# Autodesk Inventor assembly: Shoulder_support_assembly_without_mount
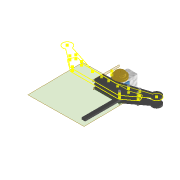
[picture p0: Inventor's stored thumbnail of the model, 180x180]
Saved by Autodesk Inventor 2022 (Build 260153000, 153)
## iProperties
Created: 2022-08-23
Part Number: Shoulder_support_assembly_without_mount
Document SubType Name: Assembly
Designer: dell
Mass: 215.1 g
Surface Area: 1120.32 cm^2
Volume: 215.1 cm^3
Author: dell
## Documents named in this file (11)
- D:\xxxx\Uni\Part IV\MECHENG_700\Part_IV_project_CAD\Bird_skeleton_prototypes\Wing_drone_V1\Bird_wing_V2\Wing_shoulder\Shoulder_support_assembly_without_mount.iam
- D:\xxxx\Uni\Part IV\MECHENG_700\Part_IV_project_CAD\Bird_skeleton_prototypes\Wing_drone_V1\Bird_wing_V2\Wing_shoulder\Vertical_bar.ipt
- D:\xxxx\Uni\Part IV\MECHENG_700\Part_IV_project_CAD\Bird_skeleton_prototypes\Wing_drone_V1\Bird_wing_V2\Wing_shoulder\Horizontal_bar_V2.ipt
- D:\xxxx\Uni\Part IV\MECHENG_700\Part_IV_project_CAD\Bird_skeleton_prototypes\Wing_drone_V1\Bird_wing_V2\Motor_pulley_assembly.iam
- D:\xxxx\Uni\Part IV\MECHENG_700\Part_IV_project_CAD\Bird_skeleton_prototypes\Wing_drone_V1\Bird_wing_V2\Wing_shoulder\Horizontal_bar_support_V2.ipt
- D:\xxxx\Uni\Part IV\MECHENG_700\Part_IV_project_CAD\Bird_skeleton_prototypes\Wing_drone_V1\Bird_wing_V2\Wing_shoulder\Horizontal_bar_spacer.ipt
- D:\xxxx\Uni\Part IV\MECHENG_700\Part_IV_project_CAD\Bird_skeleton_prototypes\Wing_drone_V1\Bird_wing_V2\Wing_shoulder\Horizontal_bar_p2_V2.ipt
- D:\xxxx\Uni\Part IV\MECHENG_700\Part_IV_project_CAD\Bird_skeleton_prototypes\Wing_drone_V1\Bird_wing_V2\Wing_shoulder\Horizontal_bar_spacer_small.ipt
- D:\xxxx\Uni\Part IV\MECHENG_700\Part_IV_project_CAD\Bird_skeleton_prototypes\Wing_drone_V1\Bird_wing_V2\M3_shoulder_bolt.ipt
- D:\xxxx\Uni\Part IV\MECHENG_700\Part_IV_project_CAD\Bird_skeleton_prototypes\Wing_drone_V1\Bird_wing_V2\M3_nut.ipt
- D:\xxxx\Uni\Part IV\MECHENG_700\Part_IV_project_CAD\Bird_skeleton_prototypes\Wing_drone_V1\Bird_wing_V2\M2.5_bolt.ipt
## Components (33 placed, 10 different names)
1. Vertical_bar:1 — Mate:5
2. Vertical_bar:4 — Mate:5, Mate:16, Mate:26, Mate:27
3. Horizontal_bar_V2:1 — Mate:16, Mate:19, Mate:20, Mate:21, Mate:23, Mate:24, Mate:25, Mate:28, Mate:30, Mate:52, Mate:53, Mate:54, Mate:55, Mate:80, Mate:81, Mate:82, Mate:83
4. Motor_pulley_assembly:3 [sub-assembly] — Mate:19, Mate:20, Mate:21, Mate:22, Mate:88, Mate:89, Mate:90, Mate:91, Mate:92, Mate:93, Mate:94, Mate:95
5. Motor_pulley_assembly:4 [sub-assembly] — Mate:23, Mate:24, Mate:25
6. Horizontal_bar_support_V2:2 — Mate:26, Mate:27, Mate:29, Mate:31, Mate:41, Mate:42, Mate:43, Mate:56, Mate:57, Mate:58, Mate:59, Mate:60, Mate:61, Mate:62, Mate:63, Mate:64, Mate:65, Mate:66, Mate:67, Mate:84, Mate:85, Mate:86, Mate:87
7. Horizontal_bar_spacer:4 — Mate:30, Mate:31
8. Horizontal_bar_spacer:5 — Mate:28, Mate:29
9. Horizontal_bar_p2_V2:1 — Mate:41, Mate:42, Mate:43, Mate:44, Mate:45, Mate:46, Mate:47, Mate:68, Mate:69, Mate:70, Mate:71, Mate:72, Mate:73, Mate:74, Mate:75
10. Horizontal_bar_spacer_small:1 — Mate:44, Mate:45
11. Horizontal_bar_spacer_small:2 — Mate:46, Mate:47
12. Horizontal_bar_spacer:6 — Mate:54, Mate:55
13. Horizontal_bar_spacer:7 — Mate:52, Mate:53
14. Horizontal_bar_spacer_small:3 — Mate:56, Mate:57
15. Horizontal_bar_spacer_small:4 — Mate:58, Mate:59
16. Horizontal_bar_spacer_small:5 — Mate:60, Mate:61
17. Horizontal_bar_spacer_small:6 — Mate:62, Mate:63
18. Horizontal_bar_spacer_small:7 — Mate:64, Mate:65
19. Horizontal_bar_spacer_small:8 — Mate:66, Mate:67
20. M3_shoulder_bolt:1 — Mate:71, Mate:73, Mate:76
21. M3_shoulder_bolt:2 — Mate:70, Mate:72, Mate:77
22. M3_shoulder_bolt:3 — Mate:69, Mate:75, Mate:78
23. M3_shoulder_bolt:4 — Mate:68, Mate:74, Mate:79
24. M3_nut:1 — Mate:77, Mate:83
25. M3_nut:2 — Mate:79, Mate:82
26. M3_nut:3 — Mate:76, Mate:81
27. M3_nut:4 — Mate:78, Mate:80
28. M3_shoulder_bolt:5 — Mate:84, Mate:86
29. M3_shoulder_bolt:6 — Mate:85, Mate:87
30. M2.5_bolt:1 — Mate:88, Mate:90
31. M2.5_bolt:2 — Mate:89, Mate:91
32. M2.5_bolt:3 — Mate:92, Mate:94
33. M2.5_bolt:4 — Mate:93, Mate:95
## Relationships (66: Mate 66)
- Mate:5 (120 mm): Vertical_bar:1 ↔ Vertical_bar:4
- Mate:16: Vertical_bar:4 ↔ Horizontal_bar_V2:1
- Mate:19: Horizontal_bar_V2:1 ↔ Motor_pulley_assembly:3
- Mate:20: Horizontal_bar_V2:1 ↔ Motor_pulley_assembly:3
- Mate:21: Horizontal_bar_V2:1 ↔ Motor_pulley_assembly:3
- Mate:22: Motor_pulley_assembly:3
- Mate:23: Horizontal_bar_V2:1 ↔ Motor_pulley_assembly:4
- Mate:24: Horizontal_bar_V2:1 ↔ Motor_pulley_assembly:4
- Mate:25: Horizontal_bar_V2:1 ↔ Motor_pulley_assembly:4
- Mate:26: Vertical_bar:4 ↔ Horizontal_bar_support_V2:2
- Mate:27: Vertical_bar:4 ↔ Horizontal_bar_support_V2:2
- Mate:28: Horizontal_bar_V2:1 ↔ Horizontal_bar_spacer:5
- Mate:29: Horizontal_bar_support_V2:2 ↔ Horizontal_bar_spacer:5
- Mate:30: Horizontal_bar_V2:1 ↔ Horizontal_bar_spacer:4
- Mate:31: Horizontal_bar_support_V2:2 ↔ Horizontal_bar_spacer:4
- Mate:41 (4.2 mm): Horizontal_bar_support_V2:2 ↔ Horizontal_bar_p2_V2:1
- Mate:42: Horizontal_bar_support_V2:2 ↔ Horizontal_bar_p2_V2:1
- Mate:43: Horizontal_bar_support_V2:2 ↔ Horizontal_bar_p2_V2:1
- Mate:44: Horizontal_bar_p2_V2:1 ↔ Horizontal_bar_spacer_small:1
- Mate:45: Horizontal_bar_p2_V2:1 ↔ Horizontal_bar_spacer_small:1
- Mate:46: Horizontal_bar_p2_V2:1 ↔ Horizontal_bar_spacer_small:2
- Mate:47: Horizontal_bar_p2_V2:1 ↔ Horizontal_bar_spacer_small:2
- Mate:52: Horizontal_bar_V2:1 ↔ Horizontal_bar_spacer:7
- Mate:53: Horizontal_bar_V2:1 ↔ Horizontal_bar_spacer:7
- Mate:54: Horizontal_bar_V2:1 ↔ Horizontal_bar_spacer:6
- Mate:55: Horizontal_bar_V2:1 ↔ Horizontal_bar_spacer:6
- Mate:56: Horizontal_bar_support_V2:2 ↔ Horizontal_bar_spacer_small:3
- Mate:57: Horizontal_bar_support_V2:2 ↔ Horizontal_bar_spacer_small:3
- Mate:58: Horizontal_bar_support_V2:2 ↔ Horizontal_bar_spacer_small:4
- Mate:59: Horizontal_bar_support_V2:2 ↔ Horizontal_bar_spacer_small:4
- Mate:60: Horizontal_bar_support_V2:2 ↔ Horizontal_bar_spacer_small:5
- Mate:61: Horizontal_bar_support_V2:2 ↔ Horizontal_bar_spacer_small:5
- Mate:62: Horizontal_bar_support_V2:2 ↔ Horizontal_bar_spacer_small:6
- Mate:63: Horizontal_bar_support_V2:2 ↔ Horizontal_bar_spacer_small:6
- Mate:64: Horizontal_bar_support_V2:2 ↔ Horizontal_bar_spacer_small:7
- Mate:65: Horizontal_bar_support_V2:2 ↔ Horizontal_bar_spacer_small:7
- Mate:66: Horizontal_bar_support_V2:2 ↔ Horizontal_bar_spacer_small:8
- Mate:67: Horizontal_bar_support_V2:2 ↔ Horizontal_bar_spacer_small:8
- Mate:68: Horizontal_bar_p2_V2:1 ↔ M3_shoulder_bolt:4
- Mate:69: Horizontal_bar_p2_V2:1 ↔ M3_shoulder_bolt:3
- Mate:70: Horizontal_bar_p2_V2:1 ↔ M3_shoulder_bolt:2
- Mate:71: Horizontal_bar_p2_V2:1 ↔ M3_shoulder_bolt:1
- Mate:72: Horizontal_bar_p2_V2:1 ↔ M3_shoulder_bolt:2
- Mate:73: Horizontal_bar_p2_V2:1 ↔ M3_shoulder_bolt:1
- Mate:74: Horizontal_bar_p2_V2:1 ↔ M3_shoulder_bolt:4
- Mate:75: Horizontal_bar_p2_V2:1 ↔ M3_shoulder_bolt:3
- Mate:76: M3_shoulder_bolt:1 ↔ M3_nut:3
- Mate:77: M3_shoulder_bolt:2 ↔ M3_nut:1
- Mate:78: M3_shoulder_bolt:3 ↔ M3_nut:4
- Mate:79: M3_shoulder_bolt:4 ↔ M3_nut:2
- Mate:80: Horizontal_bar_V2:1 ↔ M3_nut:4
- Mate:81: Horizontal_bar_V2:1 ↔ M3_nut:3
- Mate:82: Horizontal_bar_V2:1 ↔ M3_nut:2
- Mate:83: Horizontal_bar_V2:1 ↔ M3_nut:1
- Mate:84: Horizontal_bar_support_V2:2 ↔ M3_shoulder_bolt:5
- Mate:85: Horizontal_bar_support_V2:2 ↔ M3_shoulder_bolt:6
- Mate:86: Horizontal_bar_support_V2:2 ↔ M3_shoulder_bolt:5
- Mate:87: Horizontal_bar_support_V2:2 ↔ M3_shoulder_bolt:6
- Mate:88: Motor_pulley_assembly:3 ↔ M2.5_bolt:1
- Mate:89: Motor_pulley_assembly:3 ↔ M2.5_bolt:2
- Mate:90: Motor_pulley_assembly:3 ↔ M2.5_bolt:1
- Mate:91: Motor_pulley_assembly:3 ↔ M2.5_bolt:2
- Mate:92: Motor_pulley_assembly:3 ↔ M2.5_bolt:3
- Mate:93: Motor_pulley_assembly:3 ↔ M2.5_bolt:4
- Mate:94: Motor_pulley_assembly:3 ↔ M2.5_bolt:3
- Mate:95: Motor_pulley_assembly:3 ↔ M2.5_bolt:4
